# Autodesk Inventor assembly: Ensamblaje1
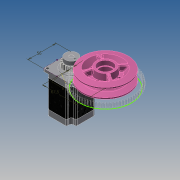
[picture p0: Inventor's stored thumbnail of the model, 180x180]
Saved by Autodesk Inventor 2017 (Build 210142000, 142)
## iProperties
Part Number: Ensamblaje1
Material: Genérico
Document SubType Name: Assembly
Designer: Leo
Author: Leo
## Documents named in this file (6)
- C:\Users\Leo\Dropbox\E\Caja Motriz\Ensamblaje1.iam
- C:\Users\Leo\Dropbox\E\Caja Motriz\esquema.ipt
- C:\Users\Leo\Dropbox\E\Caja Motriz\Piezas\Motor.ipt
- C:\Users\Leo\Dropbox\E\Caja Motriz\Transmisión\polea.ipt
- C:\Users\Leo\Dropbox\E\Caja Motriz\Ensamblaje1\Design Accelerator\Engranajes rectos1.iam
- C:\Users\Leo\Dropbox\E\Caja Motriz\Transmisión\carrete.ipt
## Components (5 placed, 5 different names)
1. esquema:1 — Nivelación:10, Nivelación:2, Nivelación:3, Coincidencia:1
2. Motor:1 — Nivelación:4, Nivelación:5, Nivelación:6, Insertar:1
3. carrete:1 — Coincidencia:1, Nivelación:8, Coincidencia:5, Coincidencia:8, Coincidencia:9
4. polea:1 — Insertar:1, Nivelación:8, Coincidencia:7, Nivelación:9
5. Engranajes rectos:1 [sub-assembly] — Coincidencia:5, Coincidencia:7, Nivelación:9, Coincidencia:8, Coincidencia:9
## Relationships (14: Flush 8, Mate 5, Insert 1)
- Nivelación:10 [Flush]: esquema:1
- Nivelación:2 [Flush]: esquema:1
- Nivelación:3 [Flush]: esquema:1
- Nivelación:4 [Flush]: Motor:1
- Nivelación:5 [Flush]: Motor:1
- Nivelación:6 [Flush]: Motor:1
- Insertar:1: Motor:1 ↔ polea:1
- Coincidencia:1 [Mate]: esquema:1 ↔ carrete:1
- Nivelación:8 [Flush]: carrete:1 ↔ polea:1
- Coincidencia:5 [Mate]: carrete:1 ↔ Engranajes rectos:1
- Coincidencia:7 [Mate]: polea:1 ↔ Engranajes rectos:1
- Nivelación:9 [Flush]: polea:1 ↔ Engranajes rectos:1
- Coincidencia:8 [Mate]: carrete:1 ↔ Engranajes rectos:1
- Coincidencia:9 [Mate]: carrete:1 ↔ Engranajes rectos:1
